# Autodesk Inventor assembly: ASY MSC 204 BELLY
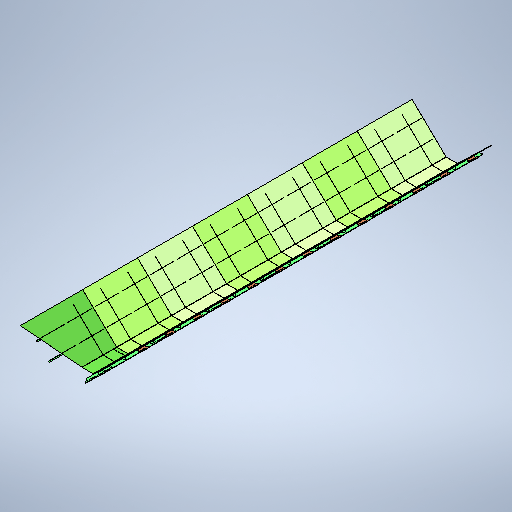
[picture p0: Inventor's stored thumbnail of the model, 512x512]
Saved by Autodesk Inventor 2025 (Build 290162010, 162A)
## iProperties
Created: 2024-07-22
Part Number: ASY MSC 204 BELLY
Document SubType Name: Assembly
Designer: pokla
Author: pokla
## Documents named in this file (5)
- C:\Users\admin\YandexDisk-badmisterfox\домашниий пк\Inventor\Manturovo\Manturovo_Se-clar\ASY MSC 204 BELLY.iam
- C:\Users\admin\YandexDisk-badmisterfox\домашниий пк\Inventor\Manturovo\Manturovo_Se-clar\MSC 041 sheet belly main.ipt
- C:\Users\admin\YandexDisk-badmisterfox\домашниий пк\Inventor\Manturovo\Manturovo_Se-clar\MSC 042 sheet belly-neck.ipt
- C:\Users\admin\YandexDisk-badmisterfox\домашниий пк\Inventor\Manturovo\Manturovo_Se-clar\MSC 067 stringer board belly.ipt
- C:\Users\admin\YandexDisk-badmisterfox\домашниий пк\Inventor\Manturovo\Manturovo_Se-clar\MSC 053 rib belly.ipt
## Components (61 placed, 6 different names)
1. MSC 041 sheet belly main.ipt:1
2. MSC 041 sheet belly main.ipt:2
3. MSC 041 sheet belly main.ipt:3
4. MSC 042 sheet belly-neck.ipt:1 — Rigid:22
5. MSC 041 sheet belly main.ipt:4
6. MSC 041 sheet belly main.ipt:5 — Rigid:22
7. MSC 041 sheet belly main.ipt:6 — Mate:4, Mate:5, Mate:6, Mate:7, Flush:1, Mate:9, Mate:10, Flush:2, Mate:11, Mate:12
8. MSC 053 rib belly.ipt:4 — Rigid:17, Rigid:20, Rigid:21, Mate:13
9. MSC 053 rib belly.ipt:3 — Rigid:18, Rigid:19, Mate:11, Mate:12, Mate:13
10. MSC 067 stringer board belly.ipt:5 — Rigid:21, Flush:2
11. MSC 067 stringer board belly.ipt:6 — Rigid:20
12. MSC 067 stringer board belly.ipt:8 — Rigid:19
13. MSC 067 stringer board belly.ipt:7 — Rigid:18
14. MSC 067 stringer board belly.ipt:2
15. MSC 067 stringer board belly.ipt:1
16. MSC 067 stringer board belly.ipt:3
17. MSC 067 stringer board belly.ipt:4
18. МОО 057 стрингер борт 7:11
19. МОО 057 стрингер борт 7:12
20. МОО 057 стрингер борт 7:13
21. МОО 057 стрингер борт 7:14
22. МОО 057 стрингер борт 7:15
23. МОО 057 стрингер борт 7:16
24. МОО 057 стрингер борт 7:17
25. МОО 057 стрингер борт 7:18
26. МОО 057 стрингер борт 7:19
27. МОО 057 стрингер борт 7:20
28. МОО 057 стрингер борт 7:21
29. МОО 057 стрингер борт 7:22
30. МОО 057 стрингер борт 7:23
31. МОО 057 стрингер борт 7:24
32. МОО 057 стрингер борт 7:25
33. МОО 057 стрингер борт 7:26
34. МОО 057 стрингер борт 7:27
35. МОО 057 стрингер борт 7:28
36. МОО 057 стрингер борт 7:29
37. МОО 057 стрингер борт 7:30
38. MSC 053 rib belly.ipt:1 — Mate:6, Mate:7, Mate:8, Rigid:17
39. MSC 053 rib belly.ipt:2 — Mate:4, Mate:5, Mate:8
40. МОО 042 шпангоут брюхо:6
41. МОО 042 шпангоут брюхо:7
42. МОО 042 шпангоут брюхо:8
43. МОО 042 шпангоут брюхо:9
44. МОО 042 шпангоут брюхо:10
45. МОО 042 шпангоут брюхо:11
46. МОО 042 шпангоут брюхо:12
47. МОО 042 шпангоут брюхо:13
48. МОО 042 шпангоут брюхо:14
49. МОО 042 шпангоут брюхо:15
50. МОО 042 шпангоут брюхо:16
51. МОО 042 шпангоут брюхо:17
52. МОО 042 шпангоут брюхо:18
53. МОО 042 шпангоут брюхо:19
54. МОО 042 шпангоут брюхо:20
55. МОО 042 шпангоут брюхо:21
56. МОО 042 шпангоут брюхо:22
57. МОО 042 шпангоут брюхо:23
58. МОО 042 шпангоут брюхо:24
59. МОО 042 шпангоут брюхо:25
60. МОО 042 шпангоут брюхо:26
61. МОО 042 шпангоут брюхо:27
## Component patterns: (6 elements, first: MSC 067 stringer board belly.ipt:2 + MSC 067 stringer board belly.ipt:1 + MSC 067 stringer board belly.ipt:3 + MSC 067 stringer board belly.ipt:4), (12 elements, first: MSC 053 rib belly.ipt:1 + MSC 053 rib belly.ipt:2)
## Relationships (27: WeldJoint 15, Mate 10, Flush 2)
- [WeldJoint]: MSC 041 sheet belly main.ipt:1 ↔ MSC 041 sheet belly main.ipt:2
- [WeldJoint]: MSC 041 sheet belly main.ipt:1 ↔ MSC 041 sheet belly main.ipt:3
- [WeldJoint]: MSC 041 sheet belly main.ipt:4 ↔ MSC 041 sheet belly main.ipt:5
- [WeldJoint]: MSC 041 sheet belly main.ipt:3 ↔ MSC 041 sheet belly main.ipt:4
- [WeldJoint]: MSC 041 sheet belly main.ipt:2 ↔ MSC 041 sheet belly main.ipt:6
- [WeldJoint]: MSC 067 stringer board belly.ipt:8 ↔ MSC 067 stringer board belly.ipt:2
- [WeldJoint]: MSC 067 stringer board belly.ipt:7 ↔ MSC 067 stringer board belly.ipt:1
- [WeldJoint]: MSC 067 stringer board belly.ipt:6 ↔ MSC 067 stringer board belly.ipt:3
- [WeldJoint]: MSC 067 stringer board belly.ipt:5 ↔ MSC 067 stringer board belly.ipt:4
- Mate:4: MSC 041 sheet belly main.ipt:6 ↔ MSC 053 rib belly.ipt:2
- Mate:5: MSC 041 sheet belly main.ipt:6 ↔ MSC 053 rib belly.ipt:2
- Mate:6: MSC 041 sheet belly main.ipt:6 ↔ MSC 053 rib belly.ipt:1
- Mate:7: MSC 041 sheet belly main.ipt:6 ↔ MSC 053 rib belly.ipt:1
- Mate:8: MSC 053 rib belly.ipt:1 ↔ MSC 053 rib belly.ipt:2
- Flush:1: MSC 041 sheet belly main.ipt:6
- Mate:9: MSC 041 sheet belly main.ipt:6
- Mate:10: MSC 041 sheet belly main.ipt:6
- Rigid:17 [WeldJoint] (480 mm): MSC 053 rib belly.ipt:4 ↔ MSC 053 rib belly.ipt:1
- Rigid:18 [WeldJoint]: MSC 053 rib belly.ipt:3 ↔ MSC 067 stringer board belly.ipt:7
- Rigid:19 [WeldJoint]: MSC 053 rib belly.ipt:3 ↔ MSC 067 stringer board belly.ipt:8
- Rigid:20 [WeldJoint]: MSC 053 rib belly.ipt:4 ↔ MSC 067 stringer board belly.ipt:6
- Rigid:21 [WeldJoint]: MSC 053 rib belly.ipt:4 ↔ MSC 067 stringer board belly.ipt:5
- Flush:2: MSC 041 sheet belly main.ipt:6 ↔ MSC 067 stringer board belly.ipt:5
- Rigid:22 [WeldJoint]: MSC 042 sheet belly-neck.ipt:1 ↔ MSC 041 sheet belly main.ipt:5
- Mate:11: MSC 041 sheet belly main.ipt:6 ↔ MSC 053 rib belly.ipt:3
- Mate:12: MSC 041 sheet belly main.ipt:6 ↔ MSC 053 rib belly.ipt:3
- Mate:13: MSC 053 rib belly.ipt:4 ↔ MSC 053 rib belly.ipt:3
